# Autodesk Inventor assembly: Hotend 2.2
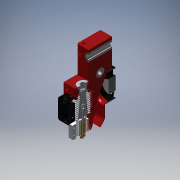
[picture p0: Inventor's stored thumbnail of the model, 180x180]
Saved by Autodesk Inventor 2018.2 (Build 222227000, 227)
## iProperties
Part Number: Hotend 2.2
Material: Generisch
Document SubType Name: Assembly
Designer: Till
Author: Till
## Documents named in this file (14)
- C:\Users\Till\Dropbox\Ultibox\ultibox\cad\Hotend 2.2.iam
- C:\Users\Till\Dropbox\Ultibox\ultibox\cad\Hotend Mount 2.2.ipt
- C:\Users\Till\Dropbox\Ultibox\ultibox\cad\E3D-HotEnd.iam
- C:\Users\Till\Dropbox\Ultibox\ultibox\cad\Clamp.ipt
- C:\Users\Till\Dropbox\Ultibox\ultibox\cad\LM6LUU.ipt
- C:\Users\Till\Dropbox\Ultibox\ultibox\cad\30mm Fan.ipt
- C:\Users\Till\Dropbox\Ultibox\ultibox\cad\fan duct 1.ipt
- C:\Users\Till\Dropbox\DIY\Stuff for other people\Sabrina\fan duct 2.ipt
- C:\Users\Till\Dropbox\Ultibox\ultibox\cad\M8 inductive probe.ipt
- C:\Users\Till\Dropbox\Ultibox\ultibox\cad\E3D Hotend\E3D-v6 1.75mm Heat Break.ipt
- C:\Users\Till\Dropbox\Ultibox\ultibox\cad\E3D Hotend\E3D-v6 Volcano Heater Block.ipt
- C:\Users\Till\Dropbox\Ultibox\ultibox\cad\E3D Hotend\E3D-v6 Volcano Nozzle.ipt
- C:\Users\Till\Dropbox\DIY\DIY Printer\Hotend UB\shroud 01 vulcan.ipt
- C:\Users\Till\Dropbox\Ultibox\ultibox\cad\40mm fan.ipt
## Components (14 placed, 13 different names)
1. Hotend Mount 2.2:1 — Passend:1, Passend:2, Fluchtend:1, Passend:3, Fluchtend:2, Fluchtend:3, Fluchtend:4, Fluchtend:5, Passend:6, Passend:7, Fluchtend:7, Fluchtend:8, Fluchtend:9, Passend:14, Passend:15, Fluchtend:10, Passend:16, Winkel:1, Fluchtend:13, Passend:22, Passend:23, Passend:24, Passend:25, Passend:26
2. E3D-HotEnd:1 [sub-assembly] — Passend:3, Fluchtend:2, Passend:19, Fluchtend:12
3. Clamp:1 — Fluchtend:3, Fluchtend:4, Fluchtend:5, Passend:8, Passend:9, Passend:10
4. LM6LUU:1 — Passend:7, Fluchtend:7
5. LM6LUU:2 — Passend:6, Fluchtend:8
6. 30mm Fan:1 — Passend:8, Passend:9, Passend:10
7. fan duct 1:1 — Fluchtend:9, Passend:14, Passend:15
8. fan duct 2:1 — Fluchtend:10
9. M8 inductive probe:1 — Passend:16, Fluchtend:11
10. E3D-v6 1.75mm Heat Break:1 — Passend:18, Passend:19, Passend:21, Fluchtend:12
11. E3D-v6 Volcano Heater Block:1 — Passend:17, Passend:18, Passend:20, Winkel:1
12. E3D-v6 Volcano Nozzle:1 — Passend:17, Passend:20, Passend:21, Fluchtend:11
13. shroud 01 vulcan:1 — Fluchtend:13, Passend:22, Passend:23
14. 40mm fan:1 — Passend:24, Passend:25, Passend:26
## Relationships (34: Mate 21, Flush 12, Angle 1)
- Passend:1 [Mate]: Hotend Mount 2.2:1
- Passend:2 [Mate]: Hotend Mount 2.2:1
- Fluchtend:1 [Flush]: Hotend Mount 2.2:1
- Passend:3 [Mate]: Hotend Mount 2.2:1 ↔ E3D-HotEnd:1
- Fluchtend:2 [Flush]: Hotend Mount 2.2:1 ↔ E3D-HotEnd:1
- Fluchtend:3 [Flush]: Hotend Mount 2.2:1 ↔ Clamp:1
- Fluchtend:4 [Flush]: Hotend Mount 2.2:1 ↔ Clamp:1
- Fluchtend:5 [Flush]: Hotend Mount 2.2:1 ↔ Clamp:1
- Passend:6 [Mate]: Hotend Mount 2.2:1 ↔ LM6LUU:2
- Passend:7 [Mate]: Hotend Mount 2.2:1 ↔ LM6LUU:1
- Fluchtend:7 [Flush]: Hotend Mount 2.2:1 ↔ LM6LUU:1
- Fluchtend:8 [Flush]: Hotend Mount 2.2:1 ↔ LM6LUU:2
- Passend:8 [Mate]: Clamp:1 ↔ 30mm Fan:1
- Passend:9 [Mate]: Clamp:1 ↔ 30mm Fan:1
- Passend:10 [Mate]: Clamp:1 ↔ 30mm Fan:1
- Fluchtend:9 [Flush]: Hotend Mount 2.2:1 ↔ fan duct 1:1
- Passend:14 [Mate] (0.25 mm): Hotend Mount 2.2:1 ↔ fan duct 1:1
- Passend:15 [Mate] (0.25 mm): Hotend Mount 2.2:1 ↔ fan duct 1:1
- Fluchtend:10 [Flush]: Hotend Mount 2.2:1 ↔ fan duct 2:1
- Passend:16 [Mate]: Hotend Mount 2.2:1 ↔ M8 inductive probe:1
- Fluchtend:11 [Flush] (1 mm): M8 inductive probe:1 ↔ E3D-v6 Volcano Nozzle:1
- Passend:17 [Mate]: E3D-v6 Volcano Heater Block:1 ↔ E3D-v6 Volcano Nozzle:1
- Passend:18 [Mate]: E3D-v6 1.75mm Heat Break:1 ↔ E3D-v6 Volcano Heater Block:1
- Passend:19 [Mate]: E3D-HotEnd:1 ↔ E3D-v6 1.75mm Heat Break:1
- Passend:20 [Mate] (1 mm): E3D-v6 Volcano Heater Block:1 ↔ E3D-v6 Volcano Nozzle:1
- Passend:21 [Mate]: E3D-v6 1.75mm Heat Break:1 ↔ E3D-v6 Volcano Nozzle:1
- Fluchtend:12 [Flush]: E3D-HotEnd:1 ↔ E3D-v6 1.75mm Heat Break:1
- Winkel:1 [Angle] (0 deg): Hotend Mount 2.2:1 ↔ E3D-v6 Volcano Heater Block:1
- Fluchtend:13 [Flush]: Hotend Mount 2.2:1 ↔ shroud 01 vulcan:1
- Passend:22 [Mate] (0.2 mm): Hotend Mount 2.2:1 ↔ shroud 01 vulcan:1
- Passend:23 [Mate] (0.2 mm): Hotend Mount 2.2:1 ↔ shroud 01 vulcan:1
- Passend:24 [Mate]: Hotend Mount 2.2:1 ↔ 40mm fan:1
- Passend:25 [Mate]: Hotend Mount 2.2:1 ↔ 40mm fan:1
- Passend:26 [Mate]: Hotend Mount 2.2:1 ↔ 40mm fan:1
